# Autodesk Inventor assembly: Ensamble eléctrico
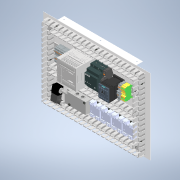
[picture p0: Inventor's stored thumbnail of the model, 180x180]
Saved by Autodesk Inventor 2021 (Build 250183000, 183)
## iProperties
Created: 2021-04-14
Part Number: Ensamble eléctrico
Document SubType Name: Assembly
Designer: Nelson
Author: Nelson
## Documents named in this file (18)
- D:\Nelson\Documentos\Inventor\PAI_ElementosInternos\Ensamble eléctrico.iam
- D:\Nelson\Documentos\Inventor\PAI_ElementosInternos\PLC-CP1E_N20DT1_D.iam
- D:\Nelson\Documentos\Inventor\PAI_ElementosInternos\FuenteDC.iam
- D:\Nelson\Documentos\Inventor\PAI_ElementosInternos\Rele de estado solido.ipt
- D:\Nelson\Documentos\Inventor\PAI_ElementosInternos\Portafusible para fusible de 2A.ipt
- D:\Nelson\Documentos\Inventor\PAI_ElementosInternos\Bobina_Electrovalvula.iam
- D:\Nelson\Documentos\Inventor\PAI_ElementosInternos\Electrovalvula-5_2.ipt
- D:\Nelson\Documentos\Inventor\PAI_ElementosInternos\Contactor.ipt
- D:\Nelson\Documentos\Inventor\PAI_ElementosInternos\Riel 35x7.5 378mm.ipt
- D:\Nelson\Documentos\Inventor\PAI_ElementosInternos\Bornera_AC.ipt
- D:\Nelson\Documentos\Inventor\PAI_ElementosInternos\Bornera_DC.ipt
- D:\Nelson\Documentos\Inventor\PAI_ElementosInternos\Bornera_Tierra.ipt
- D:\Nelson\Documentos\Inventor\PAI_ElementosInternos\Canaleta 30x30 438mm.iam
- D:\Nelson\Documentos\Inventor\PAI_ElementosInternos\Canaleta 30x30 378mm.iam
- D:\Nelson\Documentos\Inventor\PAI_ElementosInternos\Canaleta 30x30 317mm.iam
- D:\Nelson\Documentos\Inventor\PAI_ElementosInternos\Tapa_interior_1b.ipt
- D:\Nelson\Documentos\Inventor\PAI_ElementosInternos\DIN EN ISO 7049 - ST4,8 x 13 - C - H.ipt
- D:\Nelson\Documentos\Inventor\PAI_ElementosInternos\DIN EN ISO 7049 - ST4,8 x 38 - C - H.ipt
## Components (59 placed, 17 different names)
1. PLC-CP1E_N20DT1_D:1 [sub-assembly] — Mate:13, Mate:14, Mate:147, Mate:148
2. FuenteDC:1 [sub-assembly] — Mate:15, Mate:16, Mate:148, Mate:149
3. Portafusible para fusible de 2A:1 — Mate:17, Mate:18, Mate:149, Mate:150
4. Bobina_Electrovalvula:1 [sub-assembly] — Mate:9, Flush:13, Flush:14
5. Electrovalvula-5_2:1 — Mate:9, Flush:13, Flush:14, Mate:98, Mate:99, Mate:102, Flush:50, Mate:168, Mate:169, Mate:170, Mate:171
6. Contactor:1 — Mate:19, Mate:20, Mate:150, Mate:151
7. Riel 35x7.5 378mm:1 — Mate:13, Mate:14, Mate:15, Mate:16, Mate:17, Mate:18, Mate:19, Mate:20, Mate:21, Mate:22, Mate:23, Mate:24, Mate:26, Mate:27, Mate:28, Mate:29, Mate:31, Mate:32, Mate:34, Mate:35, Mate:37, Mate:38, Mate:39, Mate:40, Mate:42, Mate:43, Mate:45, Mate:46, Mate:48, Mate:49, Mate:51, Mate:52, Mate:53, Mate:54, Mate:56, Mate:57, Mate:87, Mate:96, Mate:97, Flush:45, Mate:141, Mate:143, Mate:145
8. Bornera_AC:1 — Mate:21, Mate:22, Mate:25, Mate:151
9. Bornera_AC:2 — Mate:23, Mate:24, Mate:25, Mate:65
10. Bornera_DC:1 — Mate:26, Mate:27, Mate:30, Mate:89
11. Bornera_DC:2 — Mate:28, Mate:29, Mate:30, Mate:33
12. Bornera_DC:3 — Mate:31, Mate:32, Mate:33, Mate:36
13. Bornera_DC:4 — Mate:34, Mate:35, Mate:36, Mate:146
14. Bornera_DC:5 — Mate:39, Mate:40, Mate:41, Mate:44
15. Bornera_DC:6 — Mate:42, Mate:43, Mate:44, Mate:47
16. Bornera_DC:7 — Mate:45, Mate:46, Mate:47, Mate:50
17. Bornera_DC:8 — Mate:48, Mate:49, Mate:50, Mate:89
18. Bornera_DC:9 — Mate:37, Mate:38, Mate:41, Mate:147
19. Bornera_Tierra:1 — Mate:51, Mate:52, Mate:55, Mate:65
20. Bornera_Tierra:2 — Mate:53, Mate:54, Mate:55, Mate:58
21. Bornera_Tierra:3 — Mate:56, Mate:57, Mate:58
22. Canaleta 30x30 438mm:1 [sub-assembly] — Mate:79, Mate:83, Mate:96, Flush:41, Mate:109, Flush:53, Mate:116, Mate:117, Mate:118, Mate:119, Mate:120, Mate:121
23. Canaleta 30x30 317mm:1 [sub-assembly] — Mate:79, Mate:81, Mate:87, Mate:94, Mate:99, Flush:41, Flush:42, Flush:54, Mate:110, Mate:111, Mate:112, Mate:113, Mate:114, Mate:115, Mate:146
24. Canaleta 30x30 438mm:2 [sub-assembly] — Mate:81, Mate:84, Flush:42, Flush:43, Mate:128, Mate:129, Mate:130, Mate:131, Mate:132, Mate:133
25. Canaleta 30x30 317mm:2 [sub-assembly] — Mate:83, Mate:84, Flush:43, Flush:44, Flush:45, Mate:122, Mate:123, Mate:124, Mate:125, Mate:126, Mate:127
26. Canaleta 30x30 378mm:1 [sub-assembly] — Mate:94, Mate:97, Mate:98, Mate:101, Flush:44, Flush:49, Flush:50, Mate:134, Mate:135, Mate:136, Mate:137, Mate:138, Mate:139
27. Rele de estado solido:1 — Mate:101, Mate:102, Flush:38, Mate:104, Flush:46, Flush:49, Mate:152, Mate:153, Mate:160, Mate:161
28. Rele de estado solido:2 — Flush:38, Mate:104, Flush:39, Mate:106, Flush:46, Flush:47, Mate:154, Mate:155, Mate:162, Mate:163
29. Rele de estado solido:3 — Flush:39, Mate:106, Flush:40, Mate:108, Flush:47, Flush:48, Mate:156, Mate:157, Mate:164, Mate:165
30. Rele de estado solido:4 — Flush:40, Mate:108, Flush:48, Mate:158, Mate:159, Mate:166, Mate:167
31. Tapa_interior_1b:1 — Flush:51, Flush:52, Mate:109, Flush:53, Flush:54, Mate:140, Mate:142, Mate:144
32. DIN EN ISO 7049 - C-H ST4,8 x 13 - C - H:1 — Mate:110, Mate:111
33. DIN EN ISO 7049 - C-H ST4,8 x 13 - C - H:2 — Mate:112, Mate:113
34. DIN EN ISO 7049 - C-H ST4,8 x 13 - C - H:3 — Mate:114, Mate:115
35. DIN EN ISO 7049 - C-H ST4,8 x 13 - C - H:4 — Mate:122, Mate:123
36. DIN EN ISO 7049 - C-H ST4,8 x 13 - C - H:5 — Mate:124, Mate:125
37. DIN EN ISO 7049 - C-H ST4,8 x 13 - C - H:6 — Mate:126, Mate:127
38. DIN EN ISO 7049 - C-H ST4,8 x 13 - C - H:7 — Mate:132, Mate:133
39. DIN EN ISO 7049 - C-H ST4,8 x 13 - C - H:8 — Mate:130, Mate:131
40. DIN EN ISO 7049 - C-H ST4,8 x 13 - C - H:9 — Mate:128, Mate:129
41. DIN EN ISO 7049 - C-H ST4,8 x 13 - C - H:10 — Mate:116, Mate:117
42. DIN EN ISO 7049 - C-H ST4,8 x 13 - C - H:11 — Mate:118, Mate:119
43. DIN EN ISO 7049 - C-H ST4,8 x 13 - C - H:12 — Mate:120, Mate:121
44. DIN EN ISO 7049 - C-H ST4,8 x 13 - C - H:13 — Mate:138, Mate:139
45. DIN EN ISO 7049 - C-H ST4,8 x 13 - C - H:14 — Mate:136, Mate:137
46. DIN EN ISO 7049 - C-H ST4,8 x 13 - C - H:15 — Mate:134, Mate:135
47. DIN EN ISO 7049 - C-H ST4,8 x 13 - C - H:16 — Mate:140, Mate:141
48. DIN EN ISO 7049 - C-H ST4,8 x 13 - C - H:17 — Mate:142, Mate:143
49. DIN EN ISO 7049 - C-H ST4,8 x 13 - C - H:18 — Mate:144, Mate:145
50. DIN EN ISO 7049 - C-H ST4,8 x 13 - C - H:19 — Mate:152, Mate:153
51. DIN EN ISO 7049 - C-H ST4,8 x 13 - C - H:20 — Mate:154, Mate:155
52. DIN EN ISO 7049 - C-H ST4,8 x 13 - C - H:21 — Mate:156, Mate:157
53. DIN EN ISO 7049 - C-H ST4,8 x 13 - C - H:22 — Mate:158, Mate:159
54. DIN EN ISO 7049 - C-H ST4,8 x 13 - C - H:23 — Mate:160, Mate:161
55. DIN EN ISO 7049 - C-H ST4,8 x 13 - C - H:24 — Mate:162, Mate:163
56. DIN EN ISO 7049 - C-H ST4,8 x 13 - C - H:25 — Mate:166, Mate:167
57. DIN EN ISO 7049 - C-H ST4,8 x 13 - C - H:26 — Mate:164, Mate:165
58. DIN EN ISO 7049 - C-H ST4,8 x 38 - C - H:1 — Mate:170, Mate:171
59. DIN EN ISO 7049 - C-H ST4,8 x 38 - C - H:2 — Mate:168, Mate:169
## Relationships (146: Mate 127, Flush 19)
- Mate:9: Bobina_Electrovalvula:1 ↔ Electrovalvula-5_2:1
- Flush:13: Bobina_Electrovalvula:1 ↔ Electrovalvula-5_2:1
- Flush:14: Bobina_Electrovalvula:1 ↔ Electrovalvula-5_2:1
- Mate:13: PLC-CP1E_N20DT1_D:1 ↔ Riel 35x7.5 378mm:1
- Mate:14: PLC-CP1E_N20DT1_D:1 ↔ Riel 35x7.5 378mm:1
- Mate:15: FuenteDC:1 ↔ Riel 35x7.5 378mm:1
- Mate:16: FuenteDC:1 ↔ Riel 35x7.5 378mm:1
- Mate:17: Portafusible para fusible de 2A:1 ↔ Riel 35x7.5 378mm:1
- Mate:18: Portafusible para fusible de 2A:1 ↔ Riel 35x7.5 378mm:1
- Mate:19: Contactor:1 ↔ Riel 35x7.5 378mm:1
- Mate:20: Contactor:1 ↔ Riel 35x7.5 378mm:1
- Mate:21: Riel 35x7.5 378mm:1 ↔ Bornera_AC:1
- Mate:22: Riel 35x7.5 378mm:1 ↔ Bornera_AC:1
- Mate:23: Riel 35x7.5 378mm:1 ↔ Bornera_AC:2
- Mate:24: Riel 35x7.5 378mm:1 ↔ Bornera_AC:2
- Mate:25: Bornera_AC:1 ↔ Bornera_AC:2
- Mate:26: Riel 35x7.5 378mm:1 ↔ Bornera_DC:1
- Mate:27: Riel 35x7.5 378mm:1 ↔ Bornera_DC:1
- Mate:28: Riel 35x7.5 378mm:1 ↔ Bornera_DC:2
- Mate:29: Riel 35x7.5 378mm:1 ↔ Bornera_DC:2
- Mate:30: Bornera_DC:1 ↔ Bornera_DC:2
- Mate:31: Riel 35x7.5 378mm:1 ↔ Bornera_DC:3
- Mate:32: Riel 35x7.5 378mm:1 ↔ Bornera_DC:3
- Mate:33: Bornera_DC:2 ↔ Bornera_DC:3
- Mate:34: Riel 35x7.5 378mm:1 ↔ Bornera_DC:4
- Mate:35: Riel 35x7.5 378mm:1 ↔ Bornera_DC:4
- Mate:36: Bornera_DC:3 ↔ Bornera_DC:4
- Mate:37: Riel 35x7.5 378mm:1 ↔ Bornera_DC:9
- Mate:38: Riel 35x7.5 378mm:1 ↔ Bornera_DC:9
- Mate:39: Riel 35x7.5 378mm:1 ↔ Bornera_DC:5
- Mate:40: Riel 35x7.5 378mm:1 ↔ Bornera_DC:5
- Mate:41: Bornera_DC:5 ↔ Bornera_DC:9
- Mate:42: Riel 35x7.5 378mm:1 ↔ Bornera_DC:6
- Mate:43: Riel 35x7.5 378mm:1 ↔ Bornera_DC:6
- Mate:44: Bornera_DC:5 ↔ Bornera_DC:6
- Mate:45: Riel 35x7.5 378mm:1 ↔ Bornera_DC:7
- Mate:46: Riel 35x7.5 378mm:1 ↔ Bornera_DC:7
- Mate:47: Bornera_DC:6 ↔ Bornera_DC:7
- Mate:48: Riel 35x7.5 378mm:1 ↔ Bornera_DC:8
- Mate:49: Riel 35x7.5 378mm:1 ↔ Bornera_DC:8
- Mate:50: Bornera_DC:7 ↔ Bornera_DC:8
- Mate:51: Riel 35x7.5 378mm:1 ↔ Bornera_Tierra:1
- Mate:52: Riel 35x7.5 378mm:1 ↔ Bornera_Tierra:1
- Mate:53: Riel 35x7.5 378mm:1 ↔ Bornera_Tierra:2
- Mate:54: Riel 35x7.5 378mm:1 ↔ Bornera_Tierra:2
- Mate:55: Bornera_Tierra:1 ↔ Bornera_Tierra:2
- Mate:56: Riel 35x7.5 378mm:1 ↔ Bornera_Tierra:3
- Mate:57: Riel 35x7.5 378mm:1 ↔ Bornera_Tierra:3
- Mate:58: Bornera_Tierra:2 ↔ Bornera_Tierra:3
- Mate:65 (2 mm): Bornera_AC:2 ↔ Bornera_Tierra:1
- Mate:79: Canaleta 30x30 438mm:1 ↔ Canaleta 30x30 317mm:1
- Mate:81: Canaleta 30x30 317mm:1 ↔ Canaleta 30x30 438mm:2
- Mate:83: Canaleta 30x30 438mm:1 ↔ Canaleta 30x30 317mm:2
- Mate:84: Canaleta 30x30 438mm:2 ↔ Canaleta 30x30 317mm:2
- Mate:87: Riel 35x7.5 378mm:1 ↔ Canaleta 30x30 317mm:1
- Mate:89 (2 mm): Bornera_DC:1 ↔ Bornera_DC:8
- Mate:94: Canaleta 30x30 317mm:1 ↔ Canaleta 30x30 378mm:1
- Mate:96 (47 mm): Riel 35x7.5 378mm:1 ↔ Canaleta 30x30 438mm:1
- Mate:97 (48 mm): Riel 35x7.5 378mm:1 ↔ Canaleta 30x30 378mm:1
- Mate:98 (26 mm): Electrovalvula-5_2:1 ↔ Canaleta 30x30 378mm:1
- Mate:99 (75 mm): Electrovalvula-5_2:1 ↔ Canaleta 30x30 317mm:1
- Mate:101 (23 mm): Canaleta 30x30 378mm:1 ↔ Rele de estado solido:1
- Mate:102 (10 mm): Electrovalvula-5_2:1 ↔ Rele de estado solido:1
- Flush:38: Rele de estado solido:1 ↔ Rele de estado solido:2
- Mate:104 (9 mm): Rele de estado solido:1 ↔ Rele de estado solido:2
- Flush:39: Rele de estado solido:2 ↔ Rele de estado solido:3
- Mate:106 (9 mm): Rele de estado solido:2 ↔ Rele de estado solido:3
- Flush:40: Rele de estado solido:3 ↔ Rele de estado solido:4
- Mate:108 (9 mm): Rele de estado solido:3 ↔ Rele de estado solido:4
- Flush:41: Canaleta 30x30 438mm:1 ↔ Canaleta 30x30 317mm:1
- Flush:42: Canaleta 30x30 317mm:1 ↔ Canaleta 30x30 438mm:2
- Flush:43: Canaleta 30x30 438mm:2 ↔ Canaleta 30x30 317mm:2
- Flush:44: Canaleta 30x30 317mm:2 ↔ Canaleta 30x30 378mm:1
- Flush:45: Riel 35x7.5 378mm:1 ↔ Canaleta 30x30 317mm:2
- Flush:46: Rele de estado solido:1 ↔ Rele de estado solido:2
- Flush:47: Rele de estado solido:2 ↔ Rele de estado solido:3
- Flush:48: Rele de estado solido:3 ↔ Rele de estado solido:4
- Flush:49: Canaleta 30x30 378mm:1 ↔ Rele de estado solido:1
- Flush:50: Electrovalvula-5_2:1 ↔ Canaleta 30x30 378mm:1
- Flush:51: Tapa_interior_1b:1
- Flush:52: Tapa_interior_1b:1
- Mate:109: Canaleta 30x30 438mm:1 ↔ Tapa_interior_1b:1
- Flush:53 (10.29 mm): Canaleta 30x30 438mm:1 ↔ Tapa_interior_1b:1
- Flush:54 (21 mm): Canaleta 30x30 317mm:1 ↔ Tapa_interior_1b:1
- Mate:110: Canaleta 30x30 317mm:1 ↔ DIN EN ISO 7049 - C-H ST4,8 x 13 - C - H:1
- Mate:111: Canaleta 30x30 317mm:1 ↔ DIN EN ISO 7049 - C-H ST4,8 x 13 - C - H:1
- Mate:112: Canaleta 30x30 317mm:1 ↔ DIN EN ISO 7049 - C-H ST4,8 x 13 - C - H:2
- Mate:113: Canaleta 30x30 317mm:1 ↔ DIN EN ISO 7049 - C-H ST4,8 x 13 - C - H:2
- Mate:114: Canaleta 30x30 317mm:1 ↔ DIN EN ISO 7049 - C-H ST4,8 x 13 - C - H:3
- Mate:115: Canaleta 30x30 317mm:1 ↔ DIN EN ISO 7049 - C-H ST4,8 x 13 - C - H:3
- Mate:116: Canaleta 30x30 438mm:1 ↔ DIN EN ISO 7049 - C-H ST4,8 x 13 - C - H:10
- Mate:117: Canaleta 30x30 438mm:1 ↔ DIN EN ISO 7049 - C-H ST4,8 x 13 - C - H:10
- Mate:118: Canaleta 30x30 438mm:1 ↔ DIN EN ISO 7049 - C-H ST4,8 x 13 - C - H:11
- Mate:119: Canaleta 30x30 438mm:1 ↔ DIN EN ISO 7049 - C-H ST4,8 x 13 - C - H:11
- Mate:120: Canaleta 30x30 438mm:1 ↔ DIN EN ISO 7049 - C-H ST4,8 x 13 - C - H:12
- Mate:121: Canaleta 30x30 438mm:1 ↔ DIN EN ISO 7049 - C-H ST4,8 x 13 - C - H:12
- Mate:122: Canaleta 30x30 317mm:2 ↔ DIN EN ISO 7049 - C-H ST4,8 x 13 - C - H:4
- Mate:123: Canaleta 30x30 317mm:2 ↔ DIN EN ISO 7049 - C-H ST4,8 x 13 - C - H:4
- Mate:124: Canaleta 30x30 317mm:2 ↔ DIN EN ISO 7049 - C-H ST4,8 x 13 - C - H:5
- Mate:125: Canaleta 30x30 317mm:2 ↔ DIN EN ISO 7049 - C-H ST4,8 x 13 - C - H:5
- Mate:126: Canaleta 30x30 317mm:2 ↔ DIN EN ISO 7049 - C-H ST4,8 x 13 - C - H:6
- Mate:127: Canaleta 30x30 317mm:2 ↔ DIN EN ISO 7049 - C-H ST4,8 x 13 - C - H:6
- Mate:128: Canaleta 30x30 438mm:2 ↔ DIN EN ISO 7049 - C-H ST4,8 x 13 - C - H:9
- Mate:129: Canaleta 30x30 438mm:2 ↔ DIN EN ISO 7049 - C-H ST4,8 x 13 - C - H:9
- Mate:130: Canaleta 30x30 438mm:2 ↔ DIN EN ISO 7049 - C-H ST4,8 x 13 - C - H:8
- Mate:131: Canaleta 30x30 438mm:2 ↔ DIN EN ISO 7049 - C-H ST4,8 x 13 - C - H:8
- Mate:132: Canaleta 30x30 438mm:2 ↔ DIN EN ISO 7049 - C-H ST4,8 x 13 - C - H:7
- Mate:133: Canaleta 30x30 438mm:2 ↔ DIN EN ISO 7049 - C-H ST4,8 x 13 - C - H:7
- Mate:134: Canaleta 30x30 378mm:1 ↔ DIN EN ISO 7049 - C-H ST4,8 x 13 - C - H:15
- Mate:135: Canaleta 30x30 378mm:1 ↔ DIN EN ISO 7049 - C-H ST4,8 x 13 - C - H:15
- Mate:136: Canaleta 30x30 378mm:1 ↔ DIN EN ISO 7049 - C-H ST4,8 x 13 - C - H:14
- Mate:137: Canaleta 30x30 378mm:1 ↔ DIN EN ISO 7049 - C-H ST4,8 x 13 - C - H:14
- Mate:138: Canaleta 30x30 378mm:1 ↔ DIN EN ISO 7049 - C-H ST4,8 x 13 - C - H:13
- Mate:139: Canaleta 30x30 378mm:1 ↔ DIN EN ISO 7049 - C-H ST4,8 x 13 - C - H:13
- Mate:140: Tapa_interior_1b:1 ↔ DIN EN ISO 7049 - C-H ST4,8 x 13 - C - H:16
- Mate:141: Riel 35x7.5 378mm:1 ↔ DIN EN ISO 7049 - C-H ST4,8 x 13 - C - H:16
- Mate:142: Tapa_interior_1b:1 ↔ DIN EN ISO 7049 - C-H ST4,8 x 13 - C - H:17
- Mate:143: Riel 35x7.5 378mm:1 ↔ DIN EN ISO 7049 - C-H ST4,8 x 13 - C - H:17
- Mate:144: Tapa_interior_1b:1 ↔ DIN EN ISO 7049 - C-H ST4,8 x 13 - C - H:18
- Mate:145: Riel 35x7.5 378mm:1 ↔ DIN EN ISO 7049 - C-H ST4,8 x 13 - C - H:18
- Mate:146 (35 mm): Bornera_DC:4 ↔ Canaleta 30x30 317mm:1
- Mate:147 (5 mm): PLC-CP1E_N20DT1_D:1 ↔ Bornera_DC:9
- Mate:148 (11 mm): PLC-CP1E_N20DT1_D:1 ↔ FuenteDC:1
- Mate:149 (5 mm): FuenteDC:1 ↔ Portafusible para fusible de 2A:1
- Mate:150 (5 mm): Portafusible para fusible de 2A:1 ↔ Contactor:1
- Mate:151 (5 mm): Contactor:1 ↔ Bornera_AC:1
- Mate:152: Rele de estado solido:1 ↔ DIN EN ISO 7049 - C-H ST4,8 x 13 - C - H:19
- Mate:153: Rele de estado solido:1 ↔ DIN EN ISO 7049 - C-H ST4,8 x 13 - C - H:19
- Mate:154: Rele de estado solido:2 ↔ DIN EN ISO 7049 - C-H ST4,8 x 13 - C - H:20
- Mate:155: Rele de estado solido:2 ↔ DIN EN ISO 7049 - C-H ST4,8 x 13 - C - H:20
- Mate:156: Rele de estado solido:3 ↔ DIN EN ISO 7049 - C-H ST4,8 x 13 - C - H:21
- Mate:157: Rele de estado solido:3 ↔ DIN EN ISO 7049 - C-H ST4,8 x 13 - C - H:21
- Mate:158: Rele de estado solido:4 ↔ DIN EN ISO 7049 - C-H ST4,8 x 13 - C - H:22
- Mate:159: Rele de estado solido:4 ↔ DIN EN ISO 7049 - C-H ST4,8 x 13 - C - H:22
- Mate:160: Rele de estado solido:1 ↔ DIN EN ISO 7049 - C-H ST4,8 x 13 - C - H:23
- Mate:161: Rele de estado solido:1 ↔ DIN EN ISO 7049 - C-H ST4,8 x 13 - C - H:23
- Mate:162: Rele de estado solido:2 ↔ DIN EN ISO 7049 - C-H ST4,8 x 13 - C - H:24
- Mate:163: Rele de estado solido:2 ↔ DIN EN ISO 7049 - C-H ST4,8 x 13 - C - H:24
- Mate:164: Rele de estado solido:3 ↔ DIN EN ISO 7049 - C-H ST4,8 x 13 - C - H:26
- Mate:165: Rele de estado solido:3 ↔ DIN EN ISO 7049 - C-H ST4,8 x 13 - C - H:26
- Mate:166: Rele de estado solido:4 ↔ DIN EN ISO 7049 - C-H ST4,8 x 13 - C - H:25
- Mate:167: Rele de estado solido:4 ↔ DIN EN ISO 7049 - C-H ST4,8 x 13 - C - H:25
- Mate:168: Electrovalvula-5_2:1 ↔ DIN EN ISO 7049 - C-H ST4,8 x 38 - C - H:2
- Mate:169: Electrovalvula-5_2:1 ↔ DIN EN ISO 7049 - C-H ST4,8 x 38 - C - H:2
- Mate:170: Electrovalvula-5_2:1 ↔ DIN EN ISO 7049 - C-H ST4,8 x 38 - C - H:1
- Mate:171: Electrovalvula-5_2:1 ↔ DIN EN ISO 7049 - C-H ST4,8 x 38 - C - H:1
